# Autodesk Inventor assembly: assembly
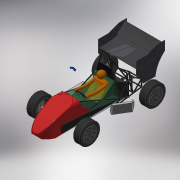
[picture p0: Inventor's stored thumbnail of the model, 180x180]
Saved by Autodesk Inventor 2018.2 (Build 222227000, 227)
## iProperties
Created: 2017-12-11
Part Number: assembly
Material: 一般
Document SubType Name: Assembly
Designer: kuwano
Author: kuwano
## Documents named in this file (4)
- D:\kuwano\Documents\Inventor\KITformula\AeroCAD2018\CAD\Inventor\製作用CAD\assembly.iam
- D:\kuwano\Documents\Inventor\KITformula\AeroCAD2018\CAD\Inventor\Assembly(KS-14.ver)\KS-14_SLow\KS-14_SLow_replace.iam
- D:\kuwano\Documents\Inventor\KITformula\AeroCAD2018\CAD\Inventor\製作用CAD\R-wing\R-wing.iam
- D:\kuwano\Documents\Inventor\KITformula\AeroCAD2018\CAD\Inventor\製作用CAD\R-wing\parts\joint\joint.iam
## Components (3 placed, 3 different names)
1. KS-14_SLow_replace:1 [sub-assembly] — メイト:1, メイト:2, メイト:3
2. R-wing:1 [sub-assembly] — フラッシュ:1
3. joint:1 [sub-assembly]
## Relationships (4: Mate 3, Flush 1)
- メイト:1 [Mate]: KS-14_SLow_replace:1
- メイト:2 [Mate]: KS-14_SLow_replace:1
- メイト:3 [Mate]: KS-14_SLow_replace:1
- フラッシュ:1 [Flush]: R-wing:1
